# Autodesk Inventor assembly: TopHopper
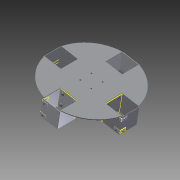
[picture p0: Inventor's stored thumbnail of the model, 180x180]
Saved by Autodesk Inventor 2013 (Build 170138000, 138)
## iProperties
Created: 2013-07-15
Part Number: TopHopper
Document SubType Name: Assembly
Designer: root
Author: root
## Documents named in this file (7)
- I:\FRC_Projects\Cad\Inventor_Projects\Shooter_No_Welding\Hopper\TopHopper.iam
- I:\FRC_Projects\Cad\Inventor_Projects\Shooter_No_Welding\Hopper\BoxWIthSUpport.iam
- I:\FRC_Projects\Cad\Inventor_Projects\Shooter_No_Welding\Hopper\SupportBAr.ipt
- I:\FRC_Projects\Cad\Inventor_Projects\Shooter_No_Welding\Hopper\BoxWIthSUpport2.iam
- I:\FRC_Projects\Cad\Inventor_Projects\Shooter_No_Welding\contentCenter\en-US\ANSI B18.5(05)\ANSI B18.5 - 1_4-20 UNC - 0.5(6).ipt
- I:\FRC_Projects\Cad\Inventor_Projects\Shooter_No_Welding\contentCenter\en-US\ANSI B18.2.2(09)\ANSI B18.2.2 - 1_4 - 20(2).ipt
- I:\FRC_Projects\Cad\Inventor_Projects\Shooter_No_Welding\Hopper\TopCover.ipt
## Components (45 placed, 6 different names)
1. Round Head Bolt - Inch 1/4-20 UNC - 0.5:1 — Mate:1, Mate:6, Mate:30, Mate:65
2. BoxWIthSUpport:1 [sub-assembly] — Mate:1, Mate:2, Mate:3, Mate:4, Mate:5, Mate:6, Mate:7, Mate:8, Flush:1, Mate:20, Mate:29, Flush:5, Mate:32
3. Round Head Bolt - Inch 1/4-20 UNC - 0.5:2 — Mate:2, Mate:8, Mate:10, Mate:68
4. Round Head Bolt - Inch 1/4-20 UNC - 0.5:3 — Mate:4, Mate:5, Mate:9, Mate:69
5. Round Head Bolt - Inch 1/4-20 UNC - 0.5:4 — Mate:3, Mate:7, Mate:33, Mate:67
6. SupportBAr:1 — Mate:9, Flush:2, Flush:3, Mate:13, Mate:16, Mate:20, Mate:72, Mate:84, Mate:90, Mate:100
7. SupportBAr:2 — Mate:10, Flush:1, Flush:2, Flush:3, Mate:11, Mate:12, Mate:14, Mate:15, Mate:70, Mate:92, Mate:99
8. SupportBAr:3 — Mate:11, Mate:12, Mate:13, Flush:4, Mate:17, Mate:19, Mate:25, Mate:31, Mate:34, Mate:48, Mate:63, Mate:79
9. SupportBAr:4 — Mate:14, Mate:15, Mate:16, Flush:4, Mate:18, Mate:26, Mate:35, Mate:36, Mate:53, Mate:64, Mate:80
10. BoxWIthSUpport2:1 [sub-assembly] — Mate:17, Mate:18, Mate:19, Mate:21, Mate:22, Mate:23, Mate:24, Mate:27, Mate:28, Mate:37, Mate:42
11. Round Head Bolt - Inch 1/4-20 UNC - 0.5:5 — Mate:22, Mate:26, Mate:60
12. Round Head Bolt - Inch 1/4-20 UNC - 0.5:6 — Mate:24, Mate:27, Mate:38, Mate:58
13. Round Head Bolt - Inch 1/4-20 UNC - 0.5:7 — Mate:21, Mate:25, Mate:59
14. Round Head Bolt - Inch 1/4-20 UNC - 0.5:8 — Mate:23, Mate:28, Mate:43, Mate:57
15. SupportBAr:5 — Mate:29, Mate:30, Flush:5, Mate:31, Flush:6, Mate:36, Mate:40, Mate:66, Mate:83, Mate:91, Mate:98, Mate:105
16. SupportBAr:6 — Mate:32, Mate:33, Flush:6, Mate:34, Mate:35, Mate:39, Mate:41, Mate:44, Mate:71, Mate:81, Mate:82, Mate:89, Mate:97, Mate:101, Mate:102, Mate:104, Mate:106, Mate:107
17. SupportBAr:7 — Mate:37, Mate:38, Mate:39, Mate:40, Mate:41, Mate:47, Mate:55, Mate:62, Mate:78, Mate:101, Mate:103
18. SupportBAr:8 — Mate:42, Mate:43, Mate:44, Mate:45, Mate:46, Mate:56, Mate:61, Mate:77
19. BoxWIthSUpport2:2 [sub-assembly] — Mate:45, Mate:46, Mate:47, Mate:48, Mate:49, Mate:50, Mate:51, Mate:52, Mate:54
20. Round Head Bolt - Inch 1/4-20 UNC - 0.5:9 — Mate:49, Mate:54, Mate:75
21. Round Head Bolt - Inch 1/4-20 UNC - 0.5:10 — Mate:50, Mate:56, Mate:73
22. Round Head Bolt - Inch 1/4-20 UNC - 0.5:11 — Mate:51, Mate:53, Mate:76
23. Round Head Bolt - Inch 1/4-20 UNC - 0.5:12 — Mate:52, Mate:55, Mate:74
24. Hex Nut - Inch 1/4 - 20:1 — Mate:73, Mate:77
25. Hex Nut - Inch 1/4 - 20:2 — Mate:67, Mate:71
26. Hex Nut - Inch 1/4 - 20:3 — Mate:69, Mate:72
27. Hex Nut - Inch 1/4 - 20:4 — Mate:59, Mate:63
28. Hex Nut - Inch 1/4 - 20:5 — Mate:74, Mate:78
29. Hex Nut - Inch 1/4 - 20:6 — Mate:68, Mate:70
30. Hex Nut - Inch 1/4 - 20:7 — Mate:65, Mate:66
31. Hex Nut - Inch 1/4 - 20:8 — Mate:58, Mate:62
32. Hex Nut - Inch 1/4 - 20:9 — Mate:75, Mate:79
33. Hex Nut - Inch 1/4 - 20:10 — Mate:76, Mate:80
34. Hex Nut - Inch 1/4 - 20:11 — Mate:60, Mate:64
35. Hex Nut - Inch 1/4 - 20:12 — Mate:57, Mate:61
36. BoxWIthSUpport:2 [sub-assembly] — Mate:81, Mate:82, Mate:83, Mate:84, Mate:85, Mate:86, Mate:87, Mate:88
37. Round Head Bolt - Inch 1/4-20 UNC - 0.5:13 — Mate:88, Mate:89, Mate:95
38. Round Head Bolt - Inch 1/4-20 UNC - 0.5:14 — Mate:85, Mate:91, Mate:93
39. Round Head Bolt - Inch 1/4-20 UNC - 0.5:15 — Mate:87, Mate:90, Mate:96
40. Round Head Bolt - Inch 1/4-20 UNC - 0.5:16 — Mate:86, Mate:92, Mate:94
41. Hex Nut - Inch 1/4 - 20:13 — Mate:93, Mate:98
42. Hex Nut - Inch 1/4 - 20:14 — Mate:96, Mate:100
43. Hex Nut - Inch 1/4 - 20:15 — Mate:94, Mate:99
44. Hex Nut - Inch 1/4 - 20:16 — Mate:95, Mate:97
45. TopCover:1 — Mate:102, Mate:103, Mate:104, Mate:105, Mate:106, Mate:107
## Relationships (113: Mate 107, Flush 6)
- Mate:1: Round Head Bolt - Inch 1/4-20 UNC - 0.5:1 ↔ BoxWIthSUpport:1
- Mate:2: BoxWIthSUpport:1 ↔ Round Head Bolt - Inch 1/4-20 UNC - 0.5:2
- Mate:3: BoxWIthSUpport:1 ↔ Round Head Bolt - Inch 1/4-20 UNC - 0.5:4
- Mate:4: BoxWIthSUpport:1 ↔ Round Head Bolt - Inch 1/4-20 UNC - 0.5:3
- Mate:5: BoxWIthSUpport:1 ↔ Round Head Bolt - Inch 1/4-20 UNC - 0.5:3
- Mate:6: Round Head Bolt - Inch 1/4-20 UNC - 0.5:1 ↔ BoxWIthSUpport:1
- Mate:7: BoxWIthSUpport:1 ↔ Round Head Bolt - Inch 1/4-20 UNC - 0.5:4
- Mate:8: BoxWIthSUpport:1 ↔ Round Head Bolt - Inch 1/4-20 UNC - 0.5:2
- Mate:9: Round Head Bolt - Inch 1/4-20 UNC - 0.5:3 ↔ SupportBAr:1
- Mate:10: Round Head Bolt - Inch 1/4-20 UNC - 0.5:2 ↔ SupportBAr:2
- Flush:1: BoxWIthSUpport:1 ↔ SupportBAr:2
- Flush:2: SupportBAr:1 ↔ SupportBAr:2
- Flush:3: SupportBAr:1 ↔ SupportBAr:2
- Mate:11: SupportBAr:2 ↔ SupportBAr:3
- Mate:12: SupportBAr:2 ↔ SupportBAr:3
- Mate:13: SupportBAr:1 ↔ SupportBAr:3
- Mate:14: SupportBAr:2 ↔ SupportBAr:4
- Mate:15: SupportBAr:2 ↔ SupportBAr:4
- Mate:16: SupportBAr:1 ↔ SupportBAr:4
- Flush:4: SupportBAr:3 ↔ SupportBAr:4
- Mate:17: SupportBAr:3 ↔ BoxWIthSUpport2:1
- Mate:18: SupportBAr:4 ↔ BoxWIthSUpport2:1
- Mate:19: SupportBAr:3 ↔ BoxWIthSUpport2:1
- Mate:20: BoxWIthSUpport:1 ↔ SupportBAr:1
- Mate:21: BoxWIthSUpport2:1 ↔ Round Head Bolt - Inch 1/4-20 UNC - 0.5:7
- Mate:22: BoxWIthSUpport2:1 ↔ Round Head Bolt - Inch 1/4-20 UNC - 0.5:5
- Mate:23: BoxWIthSUpport2:1 ↔ Round Head Bolt - Inch 1/4-20 UNC - 0.5:8
- Mate:24: BoxWIthSUpport2:1 ↔ Round Head Bolt - Inch 1/4-20 UNC - 0.5:6
- Mate:25: SupportBAr:3 ↔ Round Head Bolt - Inch 1/4-20 UNC - 0.5:7
- Mate:26: SupportBAr:4 ↔ Round Head Bolt - Inch 1/4-20 UNC - 0.5:5
- Mate:27: BoxWIthSUpport2:1 ↔ Round Head Bolt - Inch 1/4-20 UNC - 0.5:6
- Mate:28: BoxWIthSUpport2:1 ↔ Round Head Bolt - Inch 1/4-20 UNC - 0.5:8
- Mate:29: BoxWIthSUpport:1 ↔ SupportBAr:5
- Mate:30: Round Head Bolt - Inch 1/4-20 UNC - 0.5:1 ↔ SupportBAr:5
- Flush:5: BoxWIthSUpport:1 ↔ SupportBAr:5
- Mate:31: SupportBAr:3 ↔ SupportBAr:5
- Mate:32: BoxWIthSUpport:1 ↔ SupportBAr:6
- Mate:33: Round Head Bolt - Inch 1/4-20 UNC - 0.5:4 ↔ SupportBAr:6
- Flush:6: SupportBAr:5 ↔ SupportBAr:6
- Mate:34: SupportBAr:3 ↔ SupportBAr:6
- Mate:35: SupportBAr:4 ↔ SupportBAr:6
- Mate:36: SupportBAr:4 ↔ SupportBAr:5
- Mate:37: BoxWIthSUpport2:1 ↔ SupportBAr:7
- Mate:38: Round Head Bolt - Inch 1/4-20 UNC - 0.5:6 ↔ SupportBAr:7
- Mate:39: SupportBAr:6 ↔ SupportBAr:7
- Mate:40: SupportBAr:5 ↔ SupportBAr:7
- Mate:41: SupportBAr:6 ↔ SupportBAr:7
- Mate:42: BoxWIthSUpport2:1 ↔ SupportBAr:8
- Mate:43: Round Head Bolt - Inch 1/4-20 UNC - 0.5:8 ↔ SupportBAr:8
- Mate:44: SupportBAr:6 ↔ SupportBAr:8
- Mate:45: SupportBAr:8 ↔ BoxWIthSUpport2:2
- Mate:46: SupportBAr:8 ↔ BoxWIthSUpport2:2
- Mate:47: SupportBAr:7 ↔ BoxWIthSUpport2:2
- Mate:48: SupportBAr:3 ↔ BoxWIthSUpport2:2
- Mate:49: BoxWIthSUpport2:2 ↔ Round Head Bolt - Inch 1/4-20 UNC - 0.5:9
- Mate:50: BoxWIthSUpport2:2 ↔ Round Head Bolt - Inch 1/4-20 UNC - 0.5:10
- Mate:51: BoxWIthSUpport2:2 ↔ Round Head Bolt - Inch 1/4-20 UNC - 0.5:11
- Mate:52: BoxWIthSUpport2:2 ↔ Round Head Bolt - Inch 1/4-20 UNC - 0.5:12
- Mate:53: SupportBAr:4 ↔ Round Head Bolt - Inch 1/4-20 UNC - 0.5:11
- Mate:54: BoxWIthSUpport2:2 ↔ Round Head Bolt - Inch 1/4-20 UNC - 0.5:9
- Mate:55: SupportBAr:7 ↔ Round Head Bolt - Inch 1/4-20 UNC - 0.5:12
- Mate:56: SupportBAr:8 ↔ Round Head Bolt - Inch 1/4-20 UNC - 0.5:10
- Mate:57: Round Head Bolt - Inch 1/4-20 UNC - 0.5:8 ↔ Hex Nut - Inch 1/4 - 20:12
- Mate:58: Round Head Bolt - Inch 1/4-20 UNC - 0.5:6 ↔ Hex Nut - Inch 1/4 - 20:8
- Mate:59: Round Head Bolt - Inch 1/4-20 UNC - 0.5:7 ↔ Hex Nut - Inch 1/4 - 20:4
- Mate:60: Round Head Bolt - Inch 1/4-20 UNC - 0.5:5 ↔ Hex Nut - Inch 1/4 - 20:11
- Mate:61: SupportBAr:8 ↔ Hex Nut - Inch 1/4 - 20:12
- Mate:62: SupportBAr:7 ↔ Hex Nut - Inch 1/4 - 20:8
- Mate:63: SupportBAr:3 ↔ Hex Nut - Inch 1/4 - 20:4
- Mate:64: SupportBAr:4 ↔ Hex Nut - Inch 1/4 - 20:11
- Mate:65: Round Head Bolt - Inch 1/4-20 UNC - 0.5:1 ↔ Hex Nut - Inch 1/4 - 20:7
- Mate:66: SupportBAr:5 ↔ Hex Nut - Inch 1/4 - 20:7
- Mate:67: Round Head Bolt - Inch 1/4-20 UNC - 0.5:4 ↔ Hex Nut - Inch 1/4 - 20:2
- Mate:68: Round Head Bolt - Inch 1/4-20 UNC - 0.5:2 ↔ Hex Nut - Inch 1/4 - 20:6
- Mate:69: Round Head Bolt - Inch 1/4-20 UNC - 0.5:3 ↔ Hex Nut - Inch 1/4 - 20:3
- Mate:70: SupportBAr:2 ↔ Hex Nut - Inch 1/4 - 20:6
- Mate:71: SupportBAr:6 ↔ Hex Nut - Inch 1/4 - 20:2
- Mate:72: SupportBAr:1 ↔ Hex Nut - Inch 1/4 - 20:3
- Mate:73: Round Head Bolt - Inch 1/4-20 UNC - 0.5:10 ↔ Hex Nut - Inch 1/4 - 20:1
- Mate:74: Round Head Bolt - Inch 1/4-20 UNC - 0.5:12 ↔ Hex Nut - Inch 1/4 - 20:5
- Mate:75: Round Head Bolt - Inch 1/4-20 UNC - 0.5:9 ↔ Hex Nut - Inch 1/4 - 20:9
- Mate:76: Round Head Bolt - Inch 1/4-20 UNC - 0.5:11 ↔ Hex Nut - Inch 1/4 - 20:10
- Mate:77: SupportBAr:8 ↔ Hex Nut - Inch 1/4 - 20:1
- Mate:78: SupportBAr:7 ↔ Hex Nut - Inch 1/4 - 20:5
- Mate:79: SupportBAr:3 ↔ Hex Nut - Inch 1/4 - 20:9
- Mate:80: SupportBAr:4 ↔ Hex Nut - Inch 1/4 - 20:10
- Mate:81: SupportBAr:6 ↔ BoxWIthSUpport:2
- Mate:82: SupportBAr:6 ↔ BoxWIthSUpport:2
- Mate:83: SupportBAr:5 ↔ BoxWIthSUpport:2
- Mate:84: SupportBAr:1 ↔ BoxWIthSUpport:2
- Mate:85: BoxWIthSUpport:2 ↔ Round Head Bolt - Inch 1/4-20 UNC - 0.5:14
- Mate:86: BoxWIthSUpport:2 ↔ Round Head Bolt - Inch 1/4-20 UNC - 0.5:16
- Mate:87: BoxWIthSUpport:2 ↔ Round Head Bolt - Inch 1/4-20 UNC - 0.5:15
- Mate:88: BoxWIthSUpport:2 ↔ Round Head Bolt - Inch 1/4-20 UNC - 0.5:13
- Mate:89: SupportBAr:6 ↔ Round Head Bolt - Inch 1/4-20 UNC - 0.5:13
- Mate:90: SupportBAr:1 ↔ Round Head Bolt - Inch 1/4-20 UNC - 0.5:15
- Mate:91: SupportBAr:5 ↔ Round Head Bolt - Inch 1/4-20 UNC - 0.5:14
- Mate:92: SupportBAr:2 ↔ Round Head Bolt - Inch 1/4-20 UNC - 0.5:16
- Mate:93: Round Head Bolt - Inch 1/4-20 UNC - 0.5:14 ↔ Hex Nut - Inch 1/4 - 20:13
- Mate:94: Round Head Bolt - Inch 1/4-20 UNC - 0.5:16 ↔ Hex Nut - Inch 1/4 - 20:15
- Mate:95: Round Head Bolt - Inch 1/4-20 UNC - 0.5:13 ↔ Hex Nut - Inch 1/4 - 20:16
- Mate:96: Round Head Bolt - Inch 1/4-20 UNC - 0.5:15 ↔ Hex Nut - Inch 1/4 - 20:14
- Mate:97: SupportBAr:6 ↔ Hex Nut - Inch 1/4 - 20:16
- Mate:98: SupportBAr:5 ↔ Hex Nut - Inch 1/4 - 20:13
- Mate:99: SupportBAr:2 ↔ Hex Nut - Inch 1/4 - 20:15
- Mate:100: SupportBAr:1 ↔ Hex Nut - Inch 1/4 - 20:14
- Mate:101: SupportBAr:6 ↔ SupportBAr:7
- Mate:102: SupportBAr:6 ↔ TopCover:1
- Mate:103: SupportBAr:7 ↔ TopCover:1
- Mate:104: SupportBAr:6 ↔ TopCover:1
- Mate:105: SupportBAr:5 ↔ TopCover:1
- Mate:106: SupportBAr:6 ↔ TopCover:1
- Mate:107: SupportBAr:6 ↔ TopCover:1
